# Autodesk Inventor assembly: Head
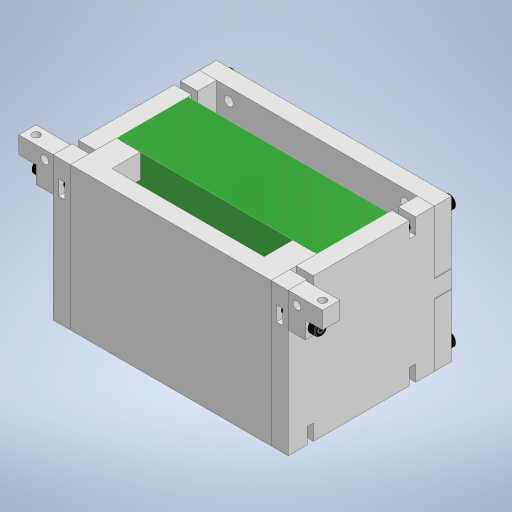
[picture p0: Inventor's stored thumbnail of the model, 512x512]
Saved by Autodesk Inventor 2024 (Build 280153000, 153)
## iProperties
Created: 2024-09-18
Part Number: Head
Document SubType Name: Assembly
Designer: Eungang
Author: Eungang
## Documents named in this file (7)
- C:\Users\Eungang\Documents\Inventor\FIGHTING_ROBOT_FINAL\부품\Head\Head.iam
- C:\Users\Eungang\Documents\Inventor\FIGHTING_ROBOT_FINAL\부품\Head\Circuit.ipt
- C:\Users\Eungang\Documents\Inventor\FIGHTING_ROBOT_FINAL\부품\Head\head_box.ipt
- C:\Users\Eungang\Documents\Inventor\FIGHTING_ROBOT_FINAL\부품\Head\head_side.ipt
- C:\Users\Eungang\Documents\Inventor\FIGHTING_ROBOT_FINAL\부품\Head\head_up.ipt
- C:\Users\Eungang\Documents\Inventor\FIGHTING_ROBOT_FINAL\부품\Head\chest_box_cap_connect.ipt
- C:\Users\Eungang\Documents\Inventor\FIGHTING_ROBOT_FINAL\부품\Bolt_Washer_Nut\CSH-ST-M2_5-15_203.ipt
## Components (13 placed, 6 different names)
1. head_box:1 — 삽입:1, 메이트:1, 메이트:2, 메이트:3
2. Circuit:1 — 삽입:1, 플러쉬:1
3. head_side:1 — 플러쉬:1, 플러쉬:2, 메이트:4, 메이트:5, 메이트:6
4. head_side:2 — 메이트:1, 메이트:2, 메이트:3, 메이트:7, 메이트:8, 메이트:9
5. head_up:1 — 플러쉬:2, 삽입:2, 삽입:3, 삽입:4, 삽입:5
6. chest_box_cap_connect:2 — 메이트:7, 메이트:8, 메이트:9, 삽입:7
7. chest_box_cap_connect:5 — 메이트:4, 메이트:5, 메이트:6, 삽입:6
8. CSH-ST-M2_5-15_203:1 — 삽입:5
9. CSH-ST-M2_5-15_203:2 — 삽입:4
10. CSH-ST-M2_5-15_203:3 — 삽입:3
11. CSH-ST-M2_5-15_203:4 — 삽입:2
12. CSH-ST-M2_5-15_203:5 — 삽입:6
13. CSH-ST-M2_5-15_203:6 — 삽입:7
## Relationships (18: Mate 9, Insert 7, Flush 2)
- 삽입:1 [Insert]: head_box:1 ↔ Circuit:1
- 플러쉬:1 [Flush]: Circuit:1 ↔ head_side:1
- 메이트:1 [Mate]: head_box:1 ↔ head_side:2
- 메이트:2 [Mate]: head_box:1 ↔ head_side:2
- 메이트:3 [Mate]: head_box:1 ↔ head_side:2
- 플러쉬:2 [Flush]: head_side:1 ↔ head_up:1
- 메이트:4 [Mate]: head_side:1 ↔ chest_box_cap_connect:5
- 메이트:5 [Mate]: head_side:1 ↔ chest_box_cap_connect:5
- 메이트:6 [Mate]: head_side:1 ↔ chest_box_cap_connect:5
- 메이트:7 [Mate]: head_side:2 ↔ chest_box_cap_connect:2
- 메이트:8 [Mate]: head_side:2 ↔ chest_box_cap_connect:2
- 메이트:9 [Mate]: head_side:2 ↔ chest_box_cap_connect:2
- 삽입:2 [Insert]: head_up:1 ↔ CSH-ST-M2_5-15_203:4
- 삽입:3 [Insert]: head_up:1 ↔ CSH-ST-M2_5-15_203:3
- 삽입:4 [Insert]: head_up:1 ↔ CSH-ST-M2_5-15_203:2
- 삽입:5 [Insert]: head_up:1 ↔ CSH-ST-M2_5-15_203:1
- 삽입:6 [Insert]: chest_box_cap_connect:5 ↔ CSH-ST-M2_5-15_203:5
- 삽입:7 [Insert]: chest_box_cap_connect:2 ↔ CSH-ST-M2_5-15_203:6
